# Autodesk Inventor assembly: xt60_mount
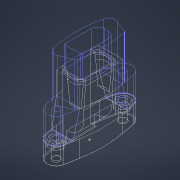
[picture p0: Inventor's stored thumbnail of the model, 180x180]
Saved by Autodesk Inventor 2022 (Build 260153000, 153)
## iProperties
Created: 2022-07-30
Part Number: xt60_mount
Document SubType Name: Assembly
Designer: ancher
Author: ancher
## Documents named in this file (3)
- E:\RC\print_3d\aos5\xt60_mount.iam
- E:\RC\print_3d\aos5\xt60_base.ipt
- E:\RC\print_3d\aos5\xt60_top.ipt
## Components (2 placed, 2 different names)
1. xt60_base:1 — Mate:1, Mate:2, Mate:3
2. xt60_top:1 — Mate:1, Mate:2, Mate:3
## Relationships (3: Mate 3)
- Mate:1: xt60_base:1 ↔ xt60_top:1
- Mate:2: xt60_base:1 ↔ xt60_top:1
- Mate:3: xt60_base:1 ↔ xt60_top:1
